# Autodesk Inventor assembly: Motor and Bracket
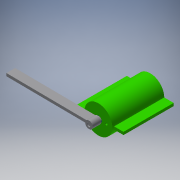
[picture p0: Inventor's stored thumbnail of the model, 180x180]
Saved by Autodesk Inventor 2016 (Build 200138000, 138)
## iProperties
Created: 2016-04-13
Part Number: Motor and Bracket
Document SubType Name: Assembly
Designer: schiu30
Author: schiu30
## Documents named in this file (4)
- C:\Users\Andrea\Documents\Dropbox\Capstone CAD\Motor + Attachment\Motor and Bracket.iam
- C:\Users\Andrea\Documents\Dropbox\Capstone CAD\Motor + Attachment\Attachment2.ipt
- C:\Users\Andrea\Documents\Dropbox\Capstone CAD\Motor + Attachment\Rotator2.ipt
- C:\Users\Andrea\Documents\Dropbox\Capstone CAD\Motor + Attachment\Motor + Shaft.iam
## Components (3 placed, 3 different names)
1. Attachment2:1 — Insert:1, Flush:1, Flush:2, Flush:3, Flush:5, Flush:6, Flush:7
2. Rotator2:1 — Flush:4, Mate:1
3. Motor + Shaft:1 [sub-assembly] — Insert:1, Flush:4, Mate:1
## Relationships (9: Flush 7, Insert 1, Mate 1)
- Insert:1: Attachment2:1 ↔ Motor + Shaft:1
- Flush:1: Attachment2:1
- Flush:2: Attachment2:1
- Flush:3: Attachment2:1
- Flush:4 (-1.016 mm): Rotator2:1 ↔ Motor + Shaft:1
- Mate:1: Rotator2:1 ↔ Motor + Shaft:1
- Flush:5: Attachment2:1
- Flush:6: Attachment2:1
- Flush:7: Attachment2:1
